# Autodesk Inventor assembly: PulleySystem 1
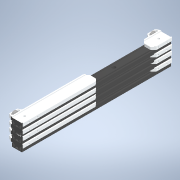
[picture p0: Inventor's stored thumbnail of the model, 180x180]
Saved by Autodesk Inventor 2020 (Build 240168000, 168)
## iProperties
Created: 2020-02-03
Part Number: PulleySystem 1
Document SubType Name: Assembly
Designer: maple
Author: maple
## Documents named in this file (2)
- C:\Users\maple\Documents\GitHub\CAD\Robotics 2019-2020\PulleySystem\PulleySystem 1.iam
- C:\Users\maple\Documents\GitHub\CAD\Robotics 2019-2020\PulleySystem\PulleySystem Part 1.ipt
## Components (4 placed, 1 different names)
1. PulleySystem Part 1:1 — Rotational:3
2. PulleySystem Part 1:2 — Rotational:2, Rotational:3
3. PulleySystem Part 1:3 — Rotational:1, Rotational:2
4. PulleySystem Part 1:4 — Rotational:1
## Relationships (3: RevoluteJoint 3)
- Rotational:1 [RevoluteJoint]: PulleySystem Part 1:3 ↔ PulleySystem Part 1:4
- Rotational:2 [RevoluteJoint]: PulleySystem Part 1:2 ↔ PulleySystem Part 1:3
- Rotational:3 [RevoluteJoint]: PulleySystem Part 1:1 ↔ PulleySystem Part 1:2
